# Autodesk Inventor assembly: Baseplate Reinforcement Assembly
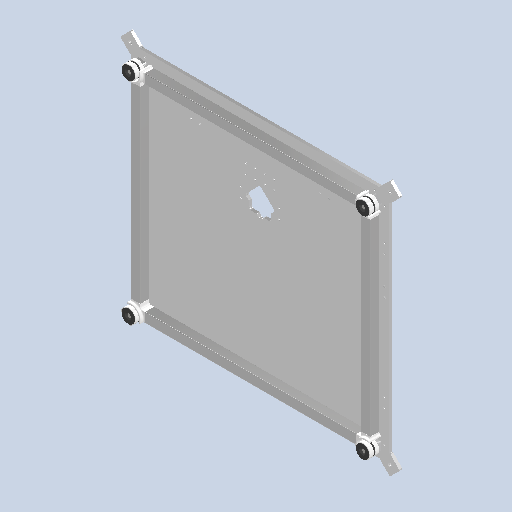
[picture p0: Inventor's stored thumbnail of the model, 512x512]
Saved by Autodesk Inventor 2024 (Build 280153000, 153)
## iProperties
Created: 2024-10-28
Part Number: Baseplate Reinforcement Assembly
Document SubType Name: Assembly
Designer: Ishaan
Author: Ishaan
## Documents named in this file (10)
- E:\Projects\Axiom--IDEX-3D-Printer\CAD\11 - Feet and Baseplate Reinforcement\Baseplate Reinforcement Assembly.iam
- E:\Projects\Axiom--IDEX-3D-Printer\CAD\02 - Frame\Printer Base Plate RevII.ipt
- E:\Projects\Axiom--IDEX-3D-Printer\CAD\00 - COTS Components\Hardware\SHCSM8x35.ipt
- E:\Projects\Axiom--IDEX-3D-Printer\CAD\11 - Feet and Baseplate Reinforcement\Levelling Foot Locknut.ipt
- E:\Projects\Axiom--IDEX-3D-Printer\CAD\11 - Feet and Baseplate Reinforcement\Levelling Foot R2.ipt
- E:\Projects\Axiom--IDEX-3D-Printer\CAD\11 - Feet and Baseplate Reinforcement\Baseplate Reinforcement Corners.ipt
- E:\Projects\Axiom--IDEX-3D-Printer\CAD\00 - COTS Components\2020 Baseplate Reinforcements\HFSC5-2020-400.ipt
- E:\Projects\Axiom--IDEX-3D-Printer\CAD\00 - COTS Components\Hardware\Low Profile M5x12.ipt
- E:\Projects\Axiom--IDEX-3D-Printer\CAD\00 - COTS Components\2020 Baseplate Reinforcements\HFSC5-2020-450.ipt
- E:\Projects\Axiom--IDEX-3D-Printer\CAD\00 - COTS Components\Hardware\M5 T SLOT NUT.ipt
## Components (69 placed, 9 different names)
1. HFSC5-2020-400:1
2. HFSC5-2020-450:2
3. HFSC5-2020-450:1
4. HFSC5-2020-400:4
5. Printer Base Plate RevII:1 — Insert:10, Insert:11, Insert:12, Insert:13, Insert:36, Insert:54, Insert:60, Insert:61, Angle:1, Insert:62, Angle:2
6. Levelling Foot R2:1
7. Levelling Foot R2:2 — Mate:6
8. Levelling Foot R2:3 — Mate:9
9. Levelling Foot R2:4
10. Levelling Foot Locknut:1 — Mate:3, Flush:3
11. Levelling Foot Locknut:2 — Mate:2, Flush:2, Flush:3
12. Levelling Foot Locknut:3 — Insert:36, Flush:1
13. Levelling Foot Locknut:4 — Mate:1, Flush:1, Flush:2
14. Baseplate Reinforcement Corners:1 — Mate:6
15. Baseplate Reinforcement Corners:2
16. Baseplate Reinforcement Corners:3 — Mate:9
17. Baseplate Reinforcement Corners:4
18. SHCSM8x35:1 — Insert:10
19. SHCSM8x35:2 — Insert:13, Mate:3
20. SHCSM8x35:3 — Insert:12, Mate:2
21. SHCSM8x35:4 — Insert:11, Mate:1
22. M5 T SLOT NUT:13 — Insert:62, Angle:2
23. M5 T SLOT NUT:14
24. M5 T SLOT NUT:15
25. M5 T SLOT NUT:16
26. M5 T SLOT NUT:17
27. M5 T SLOT NUT:18
28. M5 T SLOT NUT:19
29. M5 T SLOT NUT:20
30. M5 T SLOT NUT:21
31. M5 T SLOT NUT:22
32. M5 T SLOT NUT:23
33. M5 T SLOT NUT:24
34. M5 T SLOT NUT:1 — Insert:61, Angle:1
35. M5 T SLOT NUT:2
36. M5 T SLOT NUT:3
37. M5 T SLOT NUT:4
38. M5 T SLOT NUT:5
39. M5 T SLOT NUT:6
40. M5 T SLOT NUT:7
41. M5 T SLOT NUT:8
42. M5 T SLOT NUT:9
43. M5 T SLOT NUT:10
44. M5 T SLOT NUT:11
45. M5 T SLOT NUT:12
46. Low Profile M5x12:13 — Insert:60
47. Low Profile M5x12:14
48. Low Profile M5x12:15
49. Low Profile M5x12:16
50. Low Profile M5x12:17
51. Low Profile M5x12:18
52. Low Profile M5x12:19
53. Low Profile M5x12:20
54. Low Profile M5x12:21
55. Low Profile M5x12:22
56. Low Profile M5x12:23
57. Low Profile M5x12:24
58. Low Profile M5x12:1 — Insert:54
59. Low Profile M5x12:25
60. Low Profile M5x12:26
61. Low Profile M5x12:27
62. Low Profile M5x12:28
63. Low Profile M5x12:29
64. Low Profile M5x12:30
65. Low Profile M5x12:31
66. Low Profile M5x12:32
67. Low Profile M5x12:33
68. Low Profile M5x12:34
69. Low Profile M5x12:35
## Component patterns: (12 elements, first: M5 T SLOT NUT:13), (12 elements, first: M5 T SLOT NUT:1), (12 elements, first: Low Profile M5x12:13), (12 elements, first: Low Profile M5x12:1)
## Relationships (35: Insert 21, Mate 9, Flush 3, Angle 2)
- Insert:10: Printer Base Plate RevII:1 ↔ SHCSM8x35:1
- Insert:11: Printer Base Plate RevII:1 ↔ SHCSM8x35:4
- Insert:12: Printer Base Plate RevII:1 ↔ SHCSM8x35:3
- Insert:13: Printer Base Plate RevII:1 ↔ SHCSM8x35:2
- [Insert]: Levelling Foot R2:1 ↔ Levelling Foot Locknut:1
- [Insert]: Levelling Foot R2:2 ↔ Levelling Foot Locknut:2
- [Insert]: Levelling Foot R2:4 ↔ Levelling Foot Locknut:4
- [Insert]: Levelling Foot R2:3 ↔ Levelling Foot Locknut:3
- Insert:36 (2 mm): Printer Base Plate RevII:1 ↔ Levelling Foot Locknut:3
- Mate:1: Levelling Foot Locknut:4 ↔ SHCSM8x35:4
- Flush:1: Levelling Foot Locknut:3 ↔ Levelling Foot Locknut:4
- Mate:2: Levelling Foot Locknut:2 ↔ SHCSM8x35:3
- Flush:2: Levelling Foot Locknut:2 ↔ Levelling Foot Locknut:4
- Mate:3: Levelling Foot Locknut:1 ↔ SHCSM8x35:2
- Flush:3: Levelling Foot Locknut:1 ↔ Levelling Foot Locknut:2
- [Insert] (0.2 mm): HFSC5-2020-450:2 ↔ Baseplate Reinforcement Corners:1
- [Insert] (0.2 mm): HFSC5-2020-400:1 ↔ Baseplate Reinforcement Corners:1
- [Mate]: HFSC5-2020-450:2 ↔ Printer Base Plate RevII:1
- [Mate]: HFSC5-2020-400:1 ↔ Printer Base Plate RevII:1
- Mate:6: Levelling Foot R2:2 ↔ Baseplate Reinforcement Corners:1
- [Insert] (0.2 mm): HFSC5-2020-450:2 ↔ Baseplate Reinforcement Corners:2
- [Insert] (0.2 mm): HFSC5-2020-400:4 ↔ Baseplate Reinforcement Corners:2
- [Mate]: HFSC5-2020-400:4 ↔ Printer Base Plate RevII:1
- [Insert] (0.2 mm): HFSC5-2020-400:4 ↔ Baseplate Reinforcement Corners:3
- [Insert] (0.2 mm): HFSC5-2020-450:1 ↔ Baseplate Reinforcement Corners:3
- [Mate]: HFSC5-2020-450:1 ↔ Printer Base Plate RevII:1
- [Insert] (0.2 mm): HFSC5-2020-400:1 ↔ Baseplate Reinforcement Corners:4
- [Insert] (0.2 mm): HFSC5-2020-450:1 ↔ Baseplate Reinforcement Corners:4
- Mate:9: Levelling Foot R2:3 ↔ Baseplate Reinforcement Corners:3
- Insert:54: Printer Base Plate RevII:1 ↔ Low Profile M5x12:1
- Insert:60: Printer Base Plate RevII:1 ↔ Low Profile M5x12:13
- Insert:61 (2 mm): Printer Base Plate RevII:1 ↔ M5 T SLOT NUT:1
- Angle:1 (0 deg): Printer Base Plate RevII:1 ↔ M5 T SLOT NUT:1
- Insert:62 (2 mm): Printer Base Plate RevII:1 ↔ M5 T SLOT NUT:13
- Angle:2 (0 deg): Printer Base Plate RevII:1 ↔ M5 T SLOT NUT:13
